# Autodesk Inventor assembly: !conveyer_box
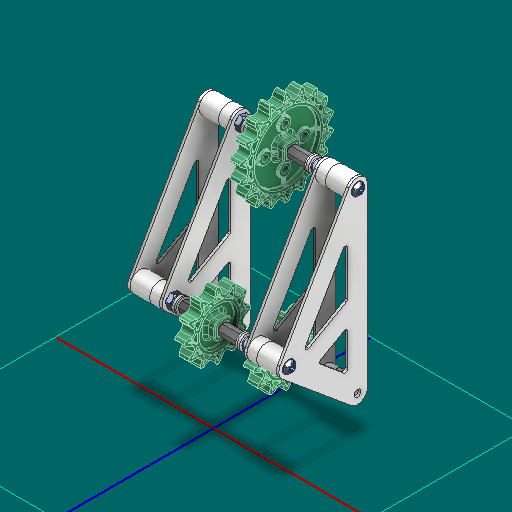
[picture p0: Inventor's stored thumbnail of the model, 512x512]
Saved by Autodesk Inventor 2025 (Build 290162000, 162)
## iProperties
Created: 2024-08-19
Part Number: !conveyer_box
Document SubType Name: Assembly
Designer: averey
Author: averey
## Documents named in this file (7)
- C:\Users\avere\vex_robotics_high_stakes\hardware\cad\ATLAS\tower\conveyer_box\!conveyer_box.iam
- C:\Users\avere\vex_robotics_high_stakes\hardware\cad\ATLAS\tower\conveyer_box\structure.iam
- structure.iam
- C:\Users\avere\vex_robotics_high_stakes\hardware\cad\ATLAS\tower\conveyer_box\structure_mirrored\structure_mirrored.iam
- C:\Users\avere\vex_robotics_high_stakes\hardware\cad\VEX-CAD-Inventor\Motion\Sprockets\9P Sprocket\9P 12T Sprocket, No Insert.iam
- C:\Users\avere\vex_robotics_high_stakes\hardware\cad\VEX-CAD-Inventor\Motion\Sprockets\9P Sprocket.iam
- C:\Users\avere\vex_robotics_high_stakes\hardware\cad\VEX-CAD-Inventor\Motion\Sprockets\9P Sprocket\9P 18T Sprocket, No Insert.iam
## Components (5 placed, 4 different names)
1. structure:1 [sub-assembly] — Insert:1, Mate:1, Mate:2, Mate:3, Insert:2, Mate:4, Insert:3
2. structure_mirrored:1 [sub-assembly] — Insert:1, Mate:1, Angle:1
3. 9P 12T Sprocket, No Insert:1 [sub-assembly] — Insert:2, Flush:1
4. 9P 12T Sprocket, No Insert:2 [sub-assembly] — Flush:1, Mate:4
5. 9P 18T Sprocket, No Insert:3 [sub-assembly] — Insert:3
## Relationships (9: Mate 4, Insert 3, Angle 1, Flush 1)
- Insert:1 (53.2035 mm): structure:1 ↔ structure_mirrored:1
- Mate:1: structure:1 ↔ structure_mirrored:1
- Mate:2: structure:1
- Mate:3 (26.6017 mm): structure:1
- Angle:1 (0 deg): structure_mirrored:1
- Insert:2: structure:1 ↔ 9P 12T Sprocket, No Insert:1
- Flush:1: 9P 12T Sprocket, No Insert:1 ↔ 9P 12T Sprocket, No Insert:2
- Mate:4: structure:1 ↔ 9P 12T Sprocket, No Insert:2
- Insert:3: structure:1 ↔ 9P 18T Sprocket, No Insert:3
